# Autodesk Inventor assembly: bed-assembly
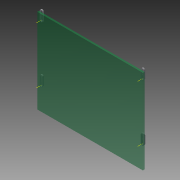
[picture p0: Inventor's stored thumbnail of the model, 180x180]
Saved by Autodesk Inventor 2015 (Build 190159000, 159)
## iProperties
Created: 2014-10-22
Part Number: bed-assembly
Document SubType Name: Assembly
Designer: caleb
Author: caleb
## Documents named in this file (4)
- C:\cygwin64\home\caleb\caleb-typea-settings\designs\simple-glass-bed\bed-assembly.iam
- C:\cygwin64\home\caleb\caleb-typea-settings\designs\simple-glass-bed\glass-print-bed.ipt
- C:\cygwin64\home\caleb\caleb-typea-settings\designs\simple-glass-bed\bed-holder.ipt
- C:\cygwin64\home\caleb\caleb-typea-settings\designs\simple-glass-bed\bed-holder-b.ipt
## Components (5 placed, 3 different names)
1. glass-print-bed:1 — Mate:1, Mate:2, Mate:3, Mate:4, Mate:5
2. bed-holder:1 — Flush:1, Mate:1, Mate:3, Flush:2
3. bed-holder-b:1 — Flush:1, Mate:2, Flush:2, Flush:5
4. bed-holder:2 — Flush:6, Mate:5
5. bed-holder-b:2 — Flush:5, Flush:6, Mate:4
## Relationships (11: Flush 6, Mate 5)
- Flush:1: bed-holder:1 ↔ bed-holder-b:1
- Mate:1: glass-print-bed:1 ↔ bed-holder:1
- Mate:2: glass-print-bed:1 ↔ bed-holder-b:1
- Mate:3: glass-print-bed:1 ↔ bed-holder:1
- Flush:2: bed-holder:1 ↔ bed-holder-b:1
- [Flush]: bed-holder:2 ↔ bed-holder-b:2
- [Flush]: bed-holder:2 ↔ bed-holder-b:2
- Flush:5: bed-holder-b:1 ↔ bed-holder-b:2
- Flush:6: bed-holder:2 ↔ bed-holder-b:2
- Mate:4: glass-print-bed:1 ↔ bed-holder-b:2
- Mate:5: glass-print-bed:1 ↔ bed-holder:2
## Named parameters: d8_d7 = 0 mm, d9_d0 = 0 mm
